# Autodesk Inventor assembly: extruder
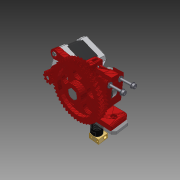
[picture p0: Inventor's stored thumbnail of the model, 180x180]
Saved by Autodesk Inventor 2014 (Build 180170000, 170)
## iProperties
Created: 2013-12-18
Part Number: extruder
Document SubType Name: Assembly
Designer: buben
Author: buben
## Documents named in this file (18)
- C:\Users\buben\Documents\GitHub\bacon\inventor files\assemblies\extruder.iam
- C:\Users\buben\Documents\GitHub\bacon\inventor files\3rd party components\j-head nozzle\Imported Components\JHead_Nozzle\JHead_Nozzle.iam
- C:\Users\buben\Documents\GitHub\bacon\inventor files\utils\hotend_mount.ipt
- C:\Users\buben\Documents\GitHub\bacon\inventor files\3rd party components\gregs wade\jonaskuehling_gregs-wade-v3_jhead-BODY-ONLY.ipt
- C:\Users\buben\Documents\GitHub\bacon\inventor files\3rd party components\nema_17_stepper\Imported Components\NEMA 17\NEMA 17.iam
- C:\Users\buben\Documents\Inventor\Content Center Files\R2014\en-US\ISO 4762(2)\ISO 4762 - M3 x 10ISO.ipt
- C:\Users\buben\Documents\GitHub\bacon\inventor files\3rd party components\gregs wade\biggearmod_fixed.ipt
- C:\Users\buben\Documents\GitHub\bacon\inventor files\3rd party components\bearing_608\Imported Components\608RS\608RS.ipt
- C:\Users\buben\Documents\GitHub\bacon\inventor files\utils\washer_m8.ipt
- C:\Users\buben\Documents\Inventor\Content Center Files\R2014\en-US\ISO 4014(1)\ISO 4014 - M8 x 55DIN EN.ipt
- C:\Users\buben\Documents\Inventor\Content Center Files\R2014\en-US\ISO 4032(2)\ISO 4032 - M8ISO.ipt
- C:\Users\buben\Documents\GitHub\bacon\inventor files\3rd party components\gregs wade\smallgearmod_fixed.ipt
- C:\Users\buben\Documents\GitHub\bacon\inventor files\3rd party components\gregs wade\jonaskuehling_gregs-wade-v3_idler-only.ipt
- C:\Users\buben\Documents\GitHub\bacon\inventor files\utils\washer_m3.ipt
- C:\Users\buben\Documents\Inventor\Content Center Files\R2014\en-US\ANSI B18.3.1M(1)\ANSI B18.3.1M - M3x0,5 x 35(2).ipt
- C:\Users\buben\Documents\Inventor\Content Center Files\R2014\en-US\ISO 7040\ISO 7040 - M3.ipt
- C:\Users\buben\Documents\GitHub\bacon\inventor files\utils\extruder_bearing_shaft.ipt
- C:\Users\buben\Documents\Inventor\Content Center Files\R2014\en-US\ANSI B18.3.1M(1)\ANSI B18.3.1M - M3x0,5 x 60(2).ipt
## Components (31 placed, 17 different names)
1. JHead_Nozzle:1 [sub-assembly] — Flush:1, Mate:1, Mate:2, Mate:3, Mate:4
2. hotend_mount:1 — Mate:3, Mate:4, Flush:2, Mate:5, Tangent:1, Tangent:2, Tangent:3
3. jonaskuehling_gregs-wade-v3_jhead-BODY-ONLY:1 — Mate:5, Tangent:1, Tangent:2, Tangent:3, Mate:6, Tangent:4, Tangent:5, Mate:7, Mate:8, Mate:9, Mate:16, Tangent:6, Tangent:7, Mate:17, Tangent:8, Tangent:9, Mate:43, Tangent:14, Tangent:15
4. NEMA 17:1 [sub-assembly] — Mate:6, Tangent:4, Tangent:5, Mate:10, Mate:11, Mate:12, Tangent:10, Tangent:11
5. ISO 4762 M3 x 10:1 — Mate:7, Mate:10
6. ISO 4762 M3 x 10:2 — Mate:8, Mate:11
7. ISO 4762 M3 x 10:3 — Mate:9, Mate:12
8. biggearmod_fixed:1 — Mate:22, Mate:23, Mate:24, Mate:25, Mate:35
9. 608RS:1 — Mate:17, Tangent:8, Tangent:9, Mate:30
10. 608RS:2 — Mate:16, Tangent:6, Tangent:7, Mate:27, Mate:28
11. CSN 02 1702 B B 8,4:1 — Mate:18, Mate:19, Mate:20, Mate:21
12. CSN 02 1702 B B 8,4:2 — Mate:18, Mate:19, Mate:28
13. CSN 02 1702 B B 8,4:3 — Mate:20, Mate:21, Mate:25, Mate:26
14. DIN EN 24014 M8 x 55:1 — Mate:22, Mate:23, Mate:24, Mate:26, Mate:27, Mate:29, Mate:32, Mate:34
15. CSN 02 1702 B B 8,4:4 — Mate:29, Mate:30, Mate:31
16. ISO 4032 M8:1 — Mate:31, Mate:32, Mate:33
17. ISO 4032 M8:2 — Mate:33, Mate:34
18. smallgearmod_fixed:1 — Tangent:10, Tangent:11, Mate:35
19. jonaskuehling_gregs-wade-v3_idler-only:1 — Mate:38, Tangent:12, Tangent:13, Mate:39, Mate:43, Mate:45, Mate:46, Tangent:16, Tangent:17, Mate:47, Mate:48, Tangent:18, Tangent:19, Tangent:20, Tangent:21, Tangent:22, Tangent:23
20. CSN 02 1702 B B 3,2:1 — Mate:48, Mate:49, Mate:50
21. CSN 02 1702 B B 3,2:2 — Insert:1, Mate:51
22. CSN 02 1702 B B 3,2:3 — Insert:2, Mate:49
23. CSN 02 1702 B B 3,2:4 — Mate:47, Mate:51, Mate:52
24. CSN 02 1702 B B 3,2:8 — Mate:39, Mate:40, Mate:41
25. CSN 02 1702 B B 3,2:9 — Mate:36, Mate:37, Mate:38
26. Broached Socket Head Cap Screw - Metric M3x0,5 x 35:1 — Mate:36, Mate:37, Tangent:12, Tangent:13, Mate:40, Mate:42, Tangent:14, Tangent:15
27. Broached Socket Head Cap Screw - Metric M3x0,5 x 60:1 — Insert:1, Mate:52, Tangent:21, Tangent:22, Tangent:23
28. Broached Socket Head Cap Screw - Metric M3x0,5 x 60:2 — Insert:2, Mate:50, Tangent:18, Tangent:19, Tangent:20
29. DIN EN ISO 7040 M3:1 — Mate:41, Mate:42
30. extruder_bearing_shaft:1 — Mate:44, Mate:45, Tangent:16, Tangent:17
31. 608RS:3 — Mate:44, Mate:46
## Relationships (76: Mate 49, Tangent 23, Flush 2, Insert 2)
- Flush:1: JHead_Nozzle:1
- Mate:1: JHead_Nozzle:1
- Mate:2: JHead_Nozzle:1
- Mate:3: JHead_Nozzle:1 ↔ hotend_mount:1
- Mate:4: JHead_Nozzle:1 ↔ hotend_mount:1
- Flush:2 (13.5 mm): hotend_mount:1
- Mate:5: hotend_mount:1 ↔ jonaskuehling_gregs-wade-v3_jhead-BODY-ONLY:1
- Tangent:1: hotend_mount:1 ↔ jonaskuehling_gregs-wade-v3_jhead-BODY-ONLY:1
- Tangent:2: hotend_mount:1 ↔ jonaskuehling_gregs-wade-v3_jhead-BODY-ONLY:1
- Tangent:3: hotend_mount:1 ↔ jonaskuehling_gregs-wade-v3_jhead-BODY-ONLY:1
- Mate:6: jonaskuehling_gregs-wade-v3_jhead-BODY-ONLY:1 ↔ NEMA 17:1
- Tangent:4: jonaskuehling_gregs-wade-v3_jhead-BODY-ONLY:1 ↔ NEMA 17:1
- Tangent:5: jonaskuehling_gregs-wade-v3_jhead-BODY-ONLY:1 ↔ NEMA 17:1
- Mate:7: jonaskuehling_gregs-wade-v3_jhead-BODY-ONLY:1 ↔ ISO 4762 M3 x 10:1
- Mate:8: jonaskuehling_gregs-wade-v3_jhead-BODY-ONLY:1 ↔ ISO 4762 M3 x 10:2
- Mate:9: jonaskuehling_gregs-wade-v3_jhead-BODY-ONLY:1 ↔ ISO 4762 M3 x 10:3
- Mate:10: NEMA 17:1 ↔ ISO 4762 M3 x 10:1
- Mate:11: NEMA 17:1 ↔ ISO 4762 M3 x 10:2
- Mate:12: NEMA 17:1 ↔ ISO 4762 M3 x 10:3
- Mate:16: jonaskuehling_gregs-wade-v3_jhead-BODY-ONLY:1 ↔ 608RS:2
- Tangent:6: jonaskuehling_gregs-wade-v3_jhead-BODY-ONLY:1 ↔ 608RS:2
- Tangent:7: jonaskuehling_gregs-wade-v3_jhead-BODY-ONLY:1 ↔ 608RS:2
- Mate:17: jonaskuehling_gregs-wade-v3_jhead-BODY-ONLY:1 ↔ 608RS:1
- Tangent:8: jonaskuehling_gregs-wade-v3_jhead-BODY-ONLY:1 ↔ 608RS:1
- Tangent:9: jonaskuehling_gregs-wade-v3_jhead-BODY-ONLY:1 ↔ 608RS:1
- Mate:18: CSN 02 1702 B B 8,4:1 ↔ CSN 02 1702 B B 8,4:2
- Mate:19: CSN 02 1702 B B 8,4:1 ↔ CSN 02 1702 B B 8,4:2
- Mate:20: CSN 02 1702 B B 8,4:1 ↔ CSN 02 1702 B B 8,4:3
- Mate:21: CSN 02 1702 B B 8,4:1 ↔ CSN 02 1702 B B 8,4:3
- Mate:22: biggearmod_fixed:1 ↔ DIN EN 24014 M8 x 55:1
- Mate:23: biggearmod_fixed:1 ↔ DIN EN 24014 M8 x 55:1
- Mate:24: biggearmod_fixed:1 ↔ DIN EN 24014 M8 x 55:1
- Mate:25: biggearmod_fixed:1 ↔ CSN 02 1702 B B 8,4:3
- Mate:26: CSN 02 1702 B B 8,4:3 ↔ DIN EN 24014 M8 x 55:1
- Mate:27: 608RS:2 ↔ DIN EN 24014 M8 x 55:1
- Mate:28: 608RS:2 ↔ CSN 02 1702 B B 8,4:2
- Mate:29: DIN EN 24014 M8 x 55:1 ↔ CSN 02 1702 B B 8,4:4
- Mate:30: 608RS:1 ↔ CSN 02 1702 B B 8,4:4
- Mate:31: CSN 02 1702 B B 8,4:4 ↔ ISO 4032 M8:1
- Mate:32: DIN EN 24014 M8 x 55:1 ↔ ISO 4032 M8:1
- Mate:33: ISO 4032 M8:1 ↔ ISO 4032 M8:2
- Mate:34: DIN EN 24014 M8 x 55:1 ↔ ISO 4032 M8:2
- Tangent:10: NEMA 17:1 ↔ smallgearmod_fixed:1
- Tangent:11: NEMA 17:1 ↔ smallgearmod_fixed:1
- Mate:35: biggearmod_fixed:1 ↔ smallgearmod_fixed:1
- Mate:36: CSN 02 1702 B B 3,2:9 ↔ Broached Socket Head Cap Screw - Metric M3x0,5 x 35:1
- Mate:37: CSN 02 1702 B B 3,2:9 ↔ Broached Socket Head Cap Screw - Metric M3x0,5 x 35:1
- Mate:38: jonaskuehling_gregs-wade-v3_idler-only:1 ↔ CSN 02 1702 B B 3,2:9
- Tangent:12: jonaskuehling_gregs-wade-v3_idler-only:1 ↔ Broached Socket Head Cap Screw - Metric M3x0,5 x 35:1
- Tangent:13: jonaskuehling_gregs-wade-v3_idler-only:1 ↔ Broached Socket Head Cap Screw - Metric M3x0,5 x 35:1
- Mate:39: jonaskuehling_gregs-wade-v3_idler-only:1 ↔ CSN 02 1702 B B 3,2:8
- Mate:40: CSN 02 1702 B B 3,2:8 ↔ Broached Socket Head Cap Screw - Metric M3x0,5 x 35:1
- Mate:41: CSN 02 1702 B B 3,2:8 ↔ DIN EN ISO 7040 M3:1
- Mate:42: Broached Socket Head Cap Screw - Metric M3x0,5 x 35:1 ↔ DIN EN ISO 7040 M3:1
- Mate:43: jonaskuehling_gregs-wade-v3_jhead-BODY-ONLY:1 ↔ jonaskuehling_gregs-wade-v3_idler-only:1
- Tangent:14: jonaskuehling_gregs-wade-v3_jhead-BODY-ONLY:1 ↔ Broached Socket Head Cap Screw - Metric M3x0,5 x 35:1
- Tangent:15: jonaskuehling_gregs-wade-v3_jhead-BODY-ONLY:1 ↔ Broached Socket Head Cap Screw - Metric M3x0,5 x 35:1
- Mate:44: extruder_bearing_shaft:1 ↔ 608RS:3
- Mate:45: jonaskuehling_gregs-wade-v3_idler-only:1 ↔ extruder_bearing_shaft:1
- Mate:46: jonaskuehling_gregs-wade-v3_idler-only:1 ↔ 608RS:3
- Tangent:16: jonaskuehling_gregs-wade-v3_idler-only:1 ↔ extruder_bearing_shaft:1
- Tangent:17: jonaskuehling_gregs-wade-v3_idler-only:1 ↔ extruder_bearing_shaft:1
- Mate:47: jonaskuehling_gregs-wade-v3_idler-only:1 ↔ CSN 02 1702 B B 3,2:4
- Mate:48: jonaskuehling_gregs-wade-v3_idler-only:1 ↔ CSN 02 1702 B B 3,2:1
- Insert:1: CSN 02 1702 B B 3,2:2 ↔ Broached Socket Head Cap Screw - Metric M3x0,5 x 60:1
- Insert:2: CSN 02 1702 B B 3,2:3 ↔ Broached Socket Head Cap Screw - Metric M3x0,5 x 60:2
- Mate:49 (15 mm): CSN 02 1702 B B 3,2:1 ↔ CSN 02 1702 B B 3,2:3
- Mate:50: CSN 02 1702 B B 3,2:1 ↔ Broached Socket Head Cap Screw - Metric M3x0,5 x 60:2
- Mate:51 (15 mm): CSN 02 1702 B B 3,2:2 ↔ CSN 02 1702 B B 3,2:4
- Mate:52: CSN 02 1702 B B 3,2:4 ↔ Broached Socket Head Cap Screw - Metric M3x0,5 x 60:1
- Tangent:18: jonaskuehling_gregs-wade-v3_idler-only:1 ↔ Broached Socket Head Cap Screw - Metric M3x0,5 x 60:2
- Tangent:19: jonaskuehling_gregs-wade-v3_idler-only:1 ↔ Broached Socket Head Cap Screw - Metric M3x0,5 x 60:2
- Tangent:20: jonaskuehling_gregs-wade-v3_idler-only:1 ↔ Broached Socket Head Cap Screw - Metric M3x0,5 x 60:2
- Tangent:21: jonaskuehling_gregs-wade-v3_idler-only:1 ↔ Broached Socket Head Cap Screw - Metric M3x0,5 x 60:1
- Tangent:22: jonaskuehling_gregs-wade-v3_idler-only:1 ↔ Broached Socket Head Cap Screw - Metric M3x0,5 x 60:1
- Tangent:23: jonaskuehling_gregs-wade-v3_idler-only:1 ↔ Broached Socket Head Cap Screw - Metric M3x0,5 x 60:1
